# Autodesk Inventor assembly: Z-Arms-OneMotor
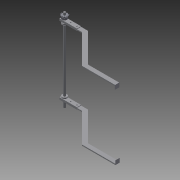
[picture p0: Inventor's stored thumbnail of the model, 180x180]
Saved by Autodesk Inventor 2013 (Build 170138000, 138)
## iProperties
Created: 2014-01-29
Part Number: Z-Arms-OneMotor
Document SubType Name: Assembly
Designer: 215152
Author: 215152
## Documents named in this file (7)
- E:\Robotics\FRC\2014\CAD\Robot\Pickup\Z-Arms-OneMotor.iam
- E:\Robotics\FRC\2014\CAD\Robot\Pickup\Z-PickupArm-R.ipt
- E:\Robotics\FRC\2014\CAD\Robot\Pickup\Z-PickupArm-L.ipt
- E:\Robotics\FRC\2014\CAD\Robot\Pickup\ArmBrace.ipt
- E:\Robotics\FRC\2014\CAD\Robot\Pickup\SuperHexagon.ipt
- E:\Robotics\FRC\2014\CAD\Robot\Pickup\Sprocket.ipt
- E:\Robotics\FRC\2014\CAD\Robot\Pickup\Bearing.ipt
## Components (10 placed, 6 different names)
1. Z-PickupArm-R:1 — Flush:1, Flush:2, Mate:1, Mate:2, Mate:3, Flush:4, Flush:5, Flush:6, Mate:6, Mate:7
2. Z-PickupArm-L:1 — Flush:1, Flush:2, Mate:1, Mate:4, Mate:5, Flush:7, Flush:8, Flush:10
3. ArmBrace:1 — Mate:3, Flush:3, Flush:4, Flush:6, Mate:11
4. ArmBrace:2 — Mate:2, Flush:3, Flush:5, Flush:11, Mate:17
5. ArmBrace:3 — Mate:4, Flush:8, Flush:9, Mate:14
6. ArmBrace:4 — Mate:5, Flush:7, Flush:9, Flush:10
7. SuperHexagon:1 — Flush:11, Mate:6, Mate:7, Mate:12, Mate:13, Mate:15, Mate:16, Mate:18, Mate:19
8. Bearing:1 — Mate:11, Mate:12, Mate:13
9. Bearing:2 — Mate:14, Mate:15, Mate:16
10. Sprocket:1 — Mate:17, Mate:18, Mate:19
## Relationships (27: Mate 16, Flush 11)
- Flush:1: Z-PickupArm-R:1 ↔ Z-PickupArm-L:1
- Flush:2: Z-PickupArm-R:1 ↔ Z-PickupArm-L:1
- Mate:1 (412.75 mm): Z-PickupArm-R:1 ↔ Z-PickupArm-L:1
- Mate:2: Z-PickupArm-R:1 ↔ ArmBrace:2
- Mate:3: Z-PickupArm-R:1 ↔ ArmBrace:1
- Mate:4: Z-PickupArm-L:1 ↔ ArmBrace:3
- Mate:5: Z-PickupArm-L:1 ↔ ArmBrace:4
- Flush:3: ArmBrace:1 ↔ ArmBrace:2
- Flush:4: Z-PickupArm-R:1 ↔ ArmBrace:1
- Flush:5: Z-PickupArm-R:1 ↔ ArmBrace:2
- Flush:6: Z-PickupArm-R:1 ↔ ArmBrace:1
- Flush:7: Z-PickupArm-L:1 ↔ ArmBrace:4
- Flush:8: Z-PickupArm-L:1 ↔ ArmBrace:3
- Flush:9: ArmBrace:3 ↔ ArmBrace:4
- Flush:10: Z-PickupArm-L:1 ↔ ArmBrace:4
- Flush:11 (-38.1 mm): ArmBrace:2 ↔ SuperHexagon:1
- Mate:6: Z-PickupArm-R:1 ↔ SuperHexagon:1
- Mate:7: Z-PickupArm-R:1 ↔ SuperHexagon:1
- Mate:11 (3.175 mm): ArmBrace:1 ↔ Bearing:1
- Mate:12: SuperHexagon:1 ↔ Bearing:1
- Mate:13: SuperHexagon:1 ↔ Bearing:1
- Mate:14 (3.175 mm): ArmBrace:3 ↔ Bearing:2
- Mate:15: SuperHexagon:1 ↔ Bearing:2
- Mate:16: SuperHexagon:1 ↔ Bearing:2
- Mate:17 (19.05 mm): ArmBrace:2 ↔ Sprocket:1
- Mate:18: SuperHexagon:1 ↔ Sprocket:1
- Mate:19: SuperHexagon:1 ↔ Sprocket:1
